# Autodesk Inventor assembly: SirHexAlotV2
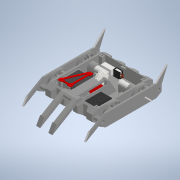
[picture p0: Inventor's stored thumbnail of the model, 180x180]
Saved by Autodesk Inventor 2020 (Build 240168000, 168)
## iProperties
Created: 2023-12-21
Part Number: SirHexAlotV2
Document SubType Name: Assembly
Designer: smz3rm
Mass: 455.578 g
Surface Area: 1715.4 cm^2
Volume: 360.282 cm^3
Density: 1.2645 g/cm^3
Author: smz3rm
## Documents named in this file (18)
- C:\Users\smz3rm\OneDrive - BP\Documents\DigitalTwin\Models\BattleBot\Flipper\SirHexAlotV2.iam
- C:\Users\smz3rm\OneDrive - BP\Documents\DigitalTwin\Models\BattleBot\Flipper\PulleyedWheelV1.ipt
- C:\Users\smz3rm\OneDrive - BP\Documents\DigitalTwin\Models\BattleBot\DriveMotorV2.ipt
- C:\Users\smz3rm\OneDrive - BP\Documents\DigitalTwin\Models\BattleBot\SwitchHolder.ipt
- C:\Users\smz3rm\OneDrive - BP\Documents\DigitalTwin\Models\BattleBot\Switch.ipt
- C:\Users\smz3rm\OneDrive - BP\Documents\DigitalTwin\Models\BattleBot\BatteryV1.ipt
- C:\Users\smz3rm\OneDrive - BP\Documents\DigitalTwin\Models\BattleBot\Flipper\Servo.ipt
- C:\Users\smz3rm\OneDrive - BP\Documents\DigitalTwin\Models\BattleBot\Flipper\PulleyedBearingWheelV1.ipt
- C:\Users\smz3rm\OneDrive - BP\Documents\DigitalTwin\Models\BattleBot\Flipper\WheelBearings.ipt
- C:\Users\smz3rm\OneDrive - BP\Documents\DigitalTwin\Models\BattleBot\Flipper\HexFlipperSpike.ipt
- C:\Users\smz3rm\OneDrive - BP\Documents\DigitalTwin\Models\BattleBot\Flipper\HexWheelGuardLeft.ipt
- C:\Users\smz3rm\OneDrive - BP\Documents\DigitalTwin\Models\BattleBot\Flipper\HexWheelGuardRight.ipt
- C:\Users\smz3rm\OneDrive - BP\Documents\DigitalTwin\Models\BattleBot\FS2A.ipt
- C:\Users\smz3rm\OneDrive - BP\Documents\DigitalTwin\Models\BattleBot\Flipper\HexBodyV2.ipt
- C:\Users\smz3rm\OneDrive - BP\Documents\DigitalTwin\Models\BattleBot\Flipper\HexFlipperV2.ipt
- C:\Users\smz3rm\OneDrive - BP\Documents\DigitalTwin\Models\BattleBot\Flipper\SirHexAlotV2\Design Accelerator\Spur Gears1.iam
- C:\Users\smz3rm\OneDrive - BP\Documents\DigitalTwin\Models\BattleBot\Flipper\ServoHornRound.ipt
- C:\Users\smz3rm\OneDrive - BP\Documents\DigitalTwin\Models\BattleBot\Flipper\HexServoCoverV2.ipt
## Components (24 placed, 17 different names)
1. HexBodyV2:1 — Mate:4, Mate:5, Mate:7, Mate:8, Mate:11, Mate:14, Mate:22, Mate:24, Mate:39, Mate:41, Mate:42, Mate:48, Flush:1, Mate:63, Mate:64, Mate:67, Mate:68, Mate:69, Mate:72, Mate:73, Mate:80, Mate:82, Flush:3, Mate:95, Mate:96, Mate:97, Mate:98, Mate:102, Mate:103, Mate:106, Mate:127, Mate:134, Mate:135, Mate:136, Mate:141, Mate:149, Mate:150, Mate:151
2. PulleyedWheelV1:1 — Mate:10, Mate:11
3. DriveMotorV2:1 — Mate:7, Mate:8, Mate:10, Mate:65, Mate:103
4. DriveMotorV2:2 — Mate:4, Mate:5, Mate:15, Mate:70, Mate:102
5. SwitchHolder:1 — Mate:19, Mate:20, Mate:21, Mate:22, Mate:95
6. Switch:1 — Mate:19, Mate:20, Mate:21
7. BatteryV1:1 — Mate:24, Mate:97, Mate:98
8. PulleyedWheelV1:5 — Mate:14, Mate:15
9. PulleyedBearingWheelV1:1 — Mate:31, Mate:32, Mate:33, Mate:42
10. PulleyedBearingWheelV1:2 — Mate:35, Mate:37, Mate:38, Mate:39, Mate:72
11. WheelBearings:1 — Mate:31, Mate:32
12. WheelBearings:2 — Mate:33, Mate:41
13. WheelBearings:3 — Mate:35
14. WheelBearings:4 — Mate:37, Mate:38
15. HexFlipperSpike:1 — Mate:93, Mate:143, Mate:144, Mate:145
16. HexFlipperSpike:2 — Mate:94, Mate:146, Mate:147, Mate:148
17. HexWheelGuardLeft:1 — Mate:63, Mate:64, Mate:65, Mate:67, Mate:92, Mate:104, Mate:105
18. HexWheelGuardRight:1 — Mate:68, Mate:69, Mate:70, Mate:73
19. FS2A:1 — Mate:80, Mate:82, Mate:96
20. Servo:1 — Mate:125, Mate:134, Mate:135, Mate:136, Mate:139, Mate:140, Mate:152
21. HexFlipperV2:1 — Mate:127, Mate:141, Rotation:1, Mate:143, Mate:144, Mate:145, Mate:146, Mate:147, Mate:148
22. Spur Gears:2 [sub-assembly] — Mate:125, Mate:142, Rotation:1
23. ServoHornRound:1 — Mate:139, Mate:140, Mate:142
24. HexServoCoverV2:1 — Mate:149, Mate:150, Mate:151, Mate:152
## Relationships (68: Mate 65, Flush 2, RelateRotation 1)
- Mate:4: HexBodyV2:1 ↔ DriveMotorV2:2
- Mate:5: HexBodyV2:1 ↔ DriveMotorV2:2
- Mate:7: HexBodyV2:1 ↔ DriveMotorV2:1
- Mate:8: HexBodyV2:1 ↔ DriveMotorV2:1
- Mate:10: PulleyedWheelV1:1 ↔ DriveMotorV2:1
- Mate:11: HexBodyV2:1 ↔ PulleyedWheelV1:1
- Mate:14: HexBodyV2:1 ↔ PulleyedWheelV1:5
- Mate:15: DriveMotorV2:2 ↔ PulleyedWheelV1:5
- Mate:19: SwitchHolder:1 ↔ Switch:1
- Mate:20: SwitchHolder:1 ↔ Switch:1
- Mate:21: SwitchHolder:1 ↔ Switch:1
- Mate:22: HexBodyV2:1 ↔ SwitchHolder:1
- Mate:24: HexBodyV2:1 ↔ BatteryV1:1
- Mate:31: PulleyedBearingWheelV1:1 ↔ WheelBearings:1
- Mate:32: PulleyedBearingWheelV1:1 ↔ WheelBearings:1
- Mate:33: PulleyedBearingWheelV1:1 ↔ WheelBearings:2
- Mate:35: PulleyedBearingWheelV1:2 ↔ WheelBearings:3
- Mate:37: PulleyedBearingWheelV1:2 ↔ WheelBearings:4
- Mate:38: PulleyedBearingWheelV1:2 ↔ WheelBearings:4
- Mate:39: HexBodyV2:1 ↔ PulleyedBearingWheelV1:2
- Mate:41: HexBodyV2:1 ↔ WheelBearings:2
- Mate:42: HexBodyV2:1 ↔ PulleyedBearingWheelV1:1
- Mate:48: HexBodyV2:1
- Flush:1: HexBodyV2:1
- Mate:63: HexBodyV2:1 ↔ HexWheelGuardLeft:1
- Mate:64: HexBodyV2:1 ↔ HexWheelGuardLeft:1
- Mate:65: DriveMotorV2:1 ↔ HexWheelGuardLeft:1
- Mate:67: HexBodyV2:1 ↔ HexWheelGuardLeft:1
- Mate:68: HexBodyV2:1 ↔ HexWheelGuardRight:1
- Mate:69: HexBodyV2:1 ↔ HexWheelGuardRight:1
- Mate:70: DriveMotorV2:2 ↔ HexWheelGuardRight:1
- Mate:72: HexBodyV2:1 ↔ PulleyedBearingWheelV1:2
- Mate:73: HexBodyV2:1 ↔ HexWheelGuardRight:1
- Mate:80: HexBodyV2:1 ↔ FS2A:1
- Mate:82: HexBodyV2:1 ↔ FS2A:1
- Flush:3: HexBodyV2:1
- Mate:92: HexWheelGuardLeft:1
- Mate:93: HexFlipperSpike:1
- Mate:94: HexFlipperSpike:2
- Mate:95: HexBodyV2:1 ↔ SwitchHolder:1
- Mate:96: HexBodyV2:1 ↔ FS2A:1
- Mate:97: HexBodyV2:1 ↔ BatteryV1:1
- Mate:98: HexBodyV2:1 ↔ BatteryV1:1
- Mate:102: HexBodyV2:1 ↔ DriveMotorV2:2
- Mate:103: HexBodyV2:1 ↔ DriveMotorV2:1
- Mate:104: HexWheelGuardLeft:1
- Mate:105: HexWheelGuardLeft:1
- Mate:106: HexBodyV2:1
- Mate:125: Servo:1 ↔ Spur Gears:2
- Mate:127: HexBodyV2:1 ↔ HexFlipperV2:1
- Mate:134: HexBodyV2:1 ↔ Servo:1
- Mate:135: HexBodyV2:1 ↔ Servo:1
- Mate:136: HexBodyV2:1 ↔ Servo:1
- Mate:139: Servo:1 ↔ ServoHornRound:1
- Mate:140: Servo:1 ↔ ServoHornRound:1
- Mate:141 (1 mm): HexBodyV2:1 ↔ HexFlipperV2:1
- Mate:142: Spur Gears:2 ↔ ServoHornRound:1
- Rotation:1 [RelateRotation] (1 ul): HexFlipperV2:1 ↔ Spur Gears:2
- Mate:143: HexFlipperSpike:1 ↔ HexFlipperV2:1
- Mate:144: HexFlipperSpike:1 ↔ HexFlipperV2:1
- Mate:145: HexFlipperSpike:1 ↔ HexFlipperV2:1
- Mate:146: HexFlipperSpike:2 ↔ HexFlipperV2:1
- Mate:147: HexFlipperSpike:2 ↔ HexFlipperV2:1
- Mate:148: HexFlipperSpike:2 ↔ HexFlipperV2:1
- Mate:149: HexBodyV2:1 ↔ HexServoCoverV2:1
- Mate:150: HexBodyV2:1 ↔ HexServoCoverV2:1
- Mate:151: HexBodyV2:1 ↔ HexServoCoverV2:1
- Mate:152: Servo:1 ↔ HexServoCoverV2:1
## Named parameters: BaseThickness = 3 mm, TopThickness = 1.778 mm, SideThickness = 4 mm, BodyWidth = 118 mm, BodyLength = 150 mm, BodyHeight = 30 mm, DriveMotorHeight = 15 mm, WheelDia = 45 mm, WheelWidth = 7 mm, WheelGrooveWidth = 5 mm, WheelGrooveDia = 18 mm, WheeGuardlSlotWidth = 15 mm, WheelPulleyDia = 2.5 mm, M3ScrewInsertBrim = 8 mm, M3ScrewDia = 3.1 mm, M3ScrewHeadDia = 6.1 mm, M3ScrewInsertDia = 4 mm, M3ScrewInsertDepth = 7 mm, DriveMotorOffset = 40 mm, DriveMotorHoleDia = 4.2 mm, M3ScrewHeadDepth = 2.2 mm, M3ScrewHeadTaper = -32.5 deg, WheelGuardScrewOffset = 7 mm, FlipperArmLength = 87.00962 mm, FlipperArmThickness = 4.6188 mm, FlipperWidth = 20 mm, WheelSpokes = 5, FlipperRodDia = 2.3 mm, FlipperMountOffset = 70 mm, FlipperMountThickness = 6 mm, FlipperSpikeWidth = 10 mm, FlipperSpikeDrop = 40.0094 mm, FlipperSpikeAngle = 30 deg, WheelGuardSpikeDrop = 37.7 mm, WheelGuardSpikeThickness = 8 mm, ServoToFlipperAxisDistance = 13.68521 mm, FlipperArmConnectorLength = 36 mm, VM3ScrewInsertDia = 3.75 mm, M2ScrewDia = 2.1 mm, WheelBearingDia = 7.15 mm, TopSupportWidth = 10 mm, TopSupportLength = 5 mm, ServoHeightOffset = 3 mm, ServoGearCount = 15, ServoGearCenterDistance = 21.29041 mm, ServoGearRatio = 1, ServoGearWidth = 10 mm, ServoToFlipperAxisAngle = 50 deg
